# Autodesk Inventor assembly: Assembly_Cube_Dichroic_Beamsplitter_25x35_v3
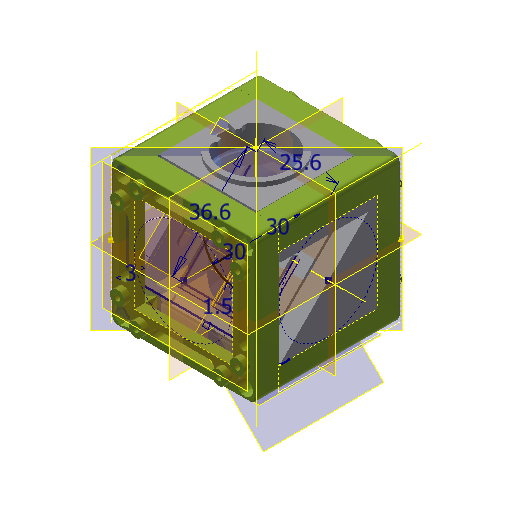
[picture p0: Inventor's stored thumbnail of the model, 512x512]
Saved by Autodesk Inventor 2022 (Build 260153000, 153)
## iProperties
Created: 2019-08-07
Part Number: Assembly_Cube_Dichroic_Beamsplitter_25x35_v3
Document SubType Name: Assembly
Designer: marsikovabarbora
Author: marsikovabarbora
## Documents named in this file (7)
- C:\Users\diederichbenedict\Dropbox\Dokumente\Promotion\PROJECTS\UC2\02_CAD\INVENTOR\uc2_v3\Assembly_Cube_Dichroic_Beamsplitter_25x35_v3.iam
- C:\Users\diederichbenedict\Dropbox\Dokumente\Promotion\PROJECTS\UC2\02_CAD\INVENTOR\uc2_v3\00_Comar_Filter_25Dia.ipt
- C:\Users\diederichbenedict\Dropbox\Dokumente\Promotion\PROJECTS\UC2\02_CAD\INVENTOR\uc2_v3\20_Cube_Insert_Beamsplittercube_Retainring_25mm.ipt
- C:\Users\diederichbenedict\Dropbox\Dokumente\Promotion\PROJECTS\UC2\02_CAD\INVENTOR\uc2_v3\20_Cube_Insert_Beamsplittercube_Base_25x35_v3.ipt
- C:\Users\diederichbenedict\Dropbox\Dokumente\Promotion\PROJECTS\UC2\02_CAD\INVENTOR\uc2_v3\00_Chroma_Dichroic_25x,3x1.ipt
- C:\Users\diederichbenedict\Dropbox\Dokumente\Promotion\PROJECTS\UC2\02_CAD\INVENTOR\uc2_v3\20_Cube_Insert_Beamsplittercube_Dichroicmirror_Retainplate_25_36.ipt
- C:\Users\diederichbenedict\Dropbox\Dokumente\Promotion\PROJECTS\UC2\02_CAD\INVENTOR\uc2_v3\Assembly_Cube_empty_IM_v3.iam
## Components (9 placed, 6 different names)
1. Assembly_Cube_empty_IM_v3:1 [sub-assembly] — Passend:12, Fluchtend:6, Fluchtend:7
2. 20_Cube_Insert_Beamsplittercube_Base_25x35_v3:1 — Insert:2, Insert:3, Insert:4, Flush:5, Mate:11, Passend:12, Fluchtend:6, Fluchtend:7, Passend:13, Passend:14, Passend:17
3. 00_Chroma_Dichroic_25x,3x1:1 — Flush:4, Passend:14, Passend:15, Passend:16
4. 00_Comar_Filter_25Dia:2 — Passend:13, Passend:17
5. 00_Comar_Filter_25Dia:3 — Insert:2
6. 20_Cube_Insert_Beamsplittercube_Retainring_25mm:1 — Insert:3, Insert:5
7. 20_Cube_Insert_Beamsplittercube_Retainring_25mm:2 — Insert:4
8. 00_Comar_Filter_25Dia:4 — Insert:5
9. 20_Cube_Insert_Beamsplittercube_Dichroicmirror_Retainplate_25_36:1 — Flush:4, Flush:5, Mate:11, Passend:15, Passend:16
## Relationships (18: Mate 8, Flush 6, Insert 4)
- [Flush]: Assembly_Cube_empty_IM_v3:1
- [Mate]: Assembly_Cube_empty_IM_v3:1
- [Flush]: Assembly_Cube_empty_IM_v3:1
- Insert:2: 20_Cube_Insert_Beamsplittercube_Base_25x35_v3:1 ↔ 00_Comar_Filter_25Dia:3
- Insert:3: 20_Cube_Insert_Beamsplittercube_Base_25x35_v3:1 ↔ 20_Cube_Insert_Beamsplittercube_Retainring_25mm:1
- Insert:4: 20_Cube_Insert_Beamsplittercube_Base_25x35_v3:1 ↔ 20_Cube_Insert_Beamsplittercube_Retainring_25mm:2
- Flush:4: 00_Chroma_Dichroic_25x,3x1:1 ↔ 20_Cube_Insert_Beamsplittercube_Dichroicmirror_Retainplate_25_36:1
- Flush:5: 20_Cube_Insert_Beamsplittercube_Base_25x35_v3:1 ↔ 20_Cube_Insert_Beamsplittercube_Dichroicmirror_Retainplate_25_36:1
- Insert:5: 20_Cube_Insert_Beamsplittercube_Retainring_25mm:1 ↔ 00_Comar_Filter_25Dia:4
- Mate:11: 20_Cube_Insert_Beamsplittercube_Base_25x35_v3:1 ↔ 20_Cube_Insert_Beamsplittercube_Dichroicmirror_Retainplate_25_36:1
- Passend:12 [Mate]: Assembly_Cube_empty_IM_v3:1 ↔ 20_Cube_Insert_Beamsplittercube_Base_25x35_v3:1
- Fluchtend:6 [Flush]: Assembly_Cube_empty_IM_v3:1 ↔ 20_Cube_Insert_Beamsplittercube_Base_25x35_v3:1
- Fluchtend:7 [Flush]: Assembly_Cube_empty_IM_v3:1 ↔ 20_Cube_Insert_Beamsplittercube_Base_25x35_v3:1
- Passend:13 [Mate]: 20_Cube_Insert_Beamsplittercube_Base_25x35_v3:1 ↔ 00_Comar_Filter_25Dia:2
- Passend:14 [Mate]: 20_Cube_Insert_Beamsplittercube_Base_25x35_v3:1 ↔ 00_Chroma_Dichroic_25x,3x1:1
- Passend:15 [Mate]: 00_Chroma_Dichroic_25x,3x1:1 ↔ 20_Cube_Insert_Beamsplittercube_Dichroicmirror_Retainplate_25_36:1
- Passend:16 [Mate]: 00_Chroma_Dichroic_25x,3x1:1 ↔ 20_Cube_Insert_Beamsplittercube_Dichroicmirror_Retainplate_25_36:1
- Passend:17 [Mate]: 20_Cube_Insert_Beamsplittercube_Base_25x35_v3:1 ↔ 00_Comar_Filter_25Dia:2
